# Autodesk Inventor assembly: AMA ROBOT #3
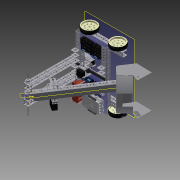
[picture p0: Inventor's stored thumbnail of the model, 180x180]
Saved by Autodesk Inventor 2014 SP2 (Build 180246200, 246)
## iProperties
Created: 2014-09-28
Part Number: AMA ROBOT #3
Document SubType Name: Assembly
Designer: Allison
Author: Allison
## Documents named in this file (19)
- C:\Users\Allison\Documents\inventor\InventorMasterProject\AMA ROBOT #3.iam
- C:\Users\Allison\Documents\Inventor\InventorMasterProject\Arm.iam
- C:\Users\Allison\Documents\Inventor\InventorMasterProject\Drivetrain.iam
- C:\Users\Allison\Documents\Inventor\InventorMasterProject\Tetrix\Channel\32mm Channel.ipt
- C:\Users\Allison\Documents\Inventor\InventorMasterProject\new.ipt
- C:\Users\Allison\Documents\Inventor\InventorMasterProject\Tetrix\Hubs and Axles\Long Axle.ipt
- C:\Users\Allison\Documents\Inventor\InventorMasterProject\Tetrix\Hubs and Axles\Axle Hub.ipt
- C:\Users\Allison\Documents\Inventor\InventorMasterProject\Tetrix\Hubs and Axles\Bronze Bushing.ipt
- C:\Users\Allison\Documents\Inventor\InventorMasterProject\Tetrix\Sprockets\16 Tooth Sprocket.ipt
- C:\Users\Allison\Documents\Inventor\InventorMasterProject\Tetrix\Spacers\Nylon Spacer 0.125in.ipt
- C:\Users\Allison\Documents\Inventor\InventorMasterProject\288mm Flat Bar-5 holes.ipt
- C:\Users\Allison\Documents\Inventor\InventorMasterProject\Tetrix\Spacers\Flower Spacer.ipt
- C:\Users\Allison\Documents\Inventor\InventorMasterProject\Tetrix\Rack and Pinion\Rack.ipt
- C:\Users\Allison\Documents\Inventor\InventorMasterProject\Tetrix\Rack and Pinion\Rack-3 Holes.ipt
- C:\Users\Allison\Documents\Inventor\InventorMasterProject\Goal Capture.iam
- C:\Users\Allison\Documents\Inventor\InventorMasterProject\Electronicsssssss.iam
- C:\Users\Allison\Documents\Inventor\InventorMasterProject\Tetrix\Standoffs\1 Inch Standoff.ipt
- C:\Users\Allison\Documents\Inventor\InventorMasterProject\Electronics Top Board.iam
- C:\Users\Allison\Documents\inventor\InventorMasterProject\box ama.ipt
## Components (31 placed, 18 different names)
1. Arm:1 [sub-assembly] — Insert:18, Insert:19, Insert:20, Insert:21, Mate:11
2. Drivetrain:1 [sub-assembly] — Insert:1, Flush:1, Flush:2, Insert:23, Insert:24, Insert:63, Insert:64, Insert:70, Insert:72, Insert:74, Insert:75, Insert:76, Flush:3
3. new:1 — Flush:2, Insert:2, Insert:7, Insert:8, Insert:14, Insert:15
4. new:2 — Insert:5, Insert:6, Insert:12, Insert:13, Insert:16, Insert:17
5. 32mm Channel:1 — Insert:7, Insert:8
6. 32mm Channel:2 — Insert:1, Flush:1, Insert:2, Insert:10, Insert:11, Insert:62
7. 32mm Channel:3 — Insert:5, Insert:6
8. 32mm Channel:4 — Insert:10, Insert:11, Insert:12, Insert:13
9. Long Axle:1 — Mate:1, Mate:2
10. Axle Hub:1 — Insert:18, Insert:19, Insert:50
11. Bronze Bushing:1 — Insert:15, Insert:57
12. Bronze Bushing:2 — Insert:14, Mate:1
13. Bronze Bushing:3 — Insert:17
14. Bronze Bushing:4 — Insert:16, Insert:50
15. Axle Hub:2 — Insert:20, Insert:21, Mate:2
16. 32mm Channel:5 — Insert:23, Insert:24
17. 16 Tooth Sprocket:1 — Insert:54, Insert:58
18. Axle Hub:9 — Insert:54
19. Nylon Spacer 0.125in:2 — Insert:57, Insert:58
20. 288mm Flat Bar-5 holes:1 — Insert:62, Insert:65, Insert:66, Insert:67, Insert:68, Insert:69, Mate:10
21. Flower Spacer:1 — Insert:63, Insert:64, Insert:65
22. Rack:1 — Insert:66, Insert:67
23. Rack-3 Holes:1 — Insert:68, Insert:69, Mate:9
24. Goal Capture:1 [sub-assembly] — Mate:9, Mate:10
25. Electronicsssssss:1 [sub-assembly] — Insert:70
26. Electronicsssssss:2 [sub-assembly] — Insert:72
27. Electronics Top Board:1 [sub-assembly]
28. 1 Inch Standoff:1 — Insert:74
29. 1 Inch Standoff:2 — Insert:75
30. 1 Inch Standoff:3 — Insert:76
31. box ama:1 — Mate:11
## Relationships (45: Insert 37, Mate 5, Flush 3)
- Insert:1: Drivetrain:1 ↔ 32mm Channel:2
- Flush:1: Drivetrain:1 ↔ 32mm Channel:2
- Flush:2: Drivetrain:1 ↔ new:1
- Insert:2: new:1 ↔ 32mm Channel:2
- Insert:5: new:2 ↔ 32mm Channel:3
- Insert:6: new:2 ↔ 32mm Channel:3
- Insert:7: new:1 ↔ 32mm Channel:1
- Insert:8: new:1 ↔ 32mm Channel:1
- Insert:10: 32mm Channel:2 ↔ 32mm Channel:4
- Insert:11: 32mm Channel:2 ↔ 32mm Channel:4
- Insert:12: new:2 ↔ 32mm Channel:4
- Insert:13: new:2 ↔ 32mm Channel:4
- Insert:14: new:1 ↔ Bronze Bushing:2
- Insert:15: new:1 ↔ Bronze Bushing:1
- Insert:16: new:2 ↔ Bronze Bushing:4
- Insert:17: new:2 ↔ Bronze Bushing:3
- Insert:18: Arm:1 ↔ Axle Hub:1
- Insert:19: Arm:1 ↔ Axle Hub:1
- Insert:20: Arm:1 ↔ Axle Hub:2
- Insert:21: Arm:1 ↔ Axle Hub:2
- Mate:1: Long Axle:1 ↔ Bronze Bushing:2
- Mate:2: Long Axle:1 ↔ Axle Hub:2
- Insert:23: Drivetrain:1 ↔ 32mm Channel:5
- Insert:24: Drivetrain:1 ↔ 32mm Channel:5
- Insert:50: Axle Hub:1 ↔ Bronze Bushing:4
- Insert:54: 16 Tooth Sprocket:1 ↔ Axle Hub:9
- Insert:57: Bronze Bushing:1 ↔ Nylon Spacer 0.125in:2
- Insert:58: 16 Tooth Sprocket:1 ↔ Nylon Spacer 0.125in:2
- Insert:62: 32mm Channel:2 ↔ 288mm Flat Bar-5 holes:1
- Insert:63: Drivetrain:1 ↔ Flower Spacer:1
- Insert:64: Drivetrain:1 ↔ Flower Spacer:1
- Insert:65: 288mm Flat Bar-5 holes:1 ↔ Flower Spacer:1
- Insert:66: 288mm Flat Bar-5 holes:1 ↔ Rack:1
- Insert:67: 288mm Flat Bar-5 holes:1 ↔ Rack:1
- Insert:68: 288mm Flat Bar-5 holes:1 ↔ Rack-3 Holes:1
- Insert:69: 288mm Flat Bar-5 holes:1 ↔ Rack-3 Holes:1
- Mate:9: Rack-3 Holes:1 ↔ Goal Capture:1
- Mate:10: 288mm Flat Bar-5 holes:1 ↔ Goal Capture:1
- Insert:70: Drivetrain:1 ↔ Electronicsssssss:1
- Insert:72: Drivetrain:1 ↔ Electronicsssssss:2
- Insert:74: Drivetrain:1 ↔ 1 Inch Standoff:1
- Insert:75: Drivetrain:1 ↔ 1 Inch Standoff:2
- Insert:76: Drivetrain:1 ↔ 1 Inch Standoff:3
- Mate:11: Arm:1 ↔ box ama:1
- Flush:3 (63.5 mm): Drivetrain:1
